# Autodesk Inventor assembly: Base Assembly
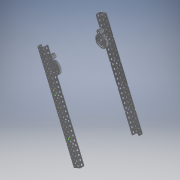
[picture p0: Inventor's stored thumbnail of the model, 180x180]
Saved by Autodesk Inventor 2018 (Build 220112000, 112)
## iProperties
Created: 2017-06-28
Part Number: Base Assembly
Document SubType Name: Assembly
Designer: James
Author: James
## Documents named in this file (4)
- C:\Users\James\Desktop\EE REU\Hardware\Vex Arm\Base Assembly.iam
- C:\Users\James\Desktop\EE REU\Hardware\Vex Arm\Vex Parts\C_Channel.ipt
- C:\Users\James\Desktop\EE REU\Hardware\Vex Arm\Vex Parts\12 Tooth Metal Pinion.ipt
- C:\Users\James\Desktop\EE REU\Hardware\Vex Arm\Vex Parts\Vex Gear Kit\VEX-36-TOOTH-GEAR.ipt
## Components (6 placed, 3 different names)
1. C_Channel:3 — Flush:1, Mate:1, Flush:2, Insert:2, Insert:4
2. C_Channel:4 — Flush:1, Mate:1, Flush:2, Insert:3, Insert:5
3. 12 Tooth Metal Pinion:2 — Insert:2
4. 12 Tooth Metal Pinion:3 — Insert:5
5. VEX-36-TOOTH-GEAR:1 — Insert:3
6. VEX-36-TOOTH-GEAR:2 — Insert:4
## Relationships (7: Insert 4, Flush 2, Mate 1)
- Flush:1: C_Channel:3 ↔ C_Channel:4
- Mate:1 (200 mm): C_Channel:3 ↔ C_Channel:4
- Flush:2: C_Channel:3 ↔ C_Channel:4
- Insert:2 (17 mm): C_Channel:3 ↔ 12 Tooth Metal Pinion:2
- Insert:3 (20 mm): C_Channel:4 ↔ VEX-36-TOOTH-GEAR:1
- Insert:4 (20 mm): C_Channel:3 ↔ VEX-36-TOOTH-GEAR:2
- Insert:5 (20 mm): C_Channel:4 ↔ 12 Tooth Metal Pinion:3
